# Autodesk Inventor assembly: 100008
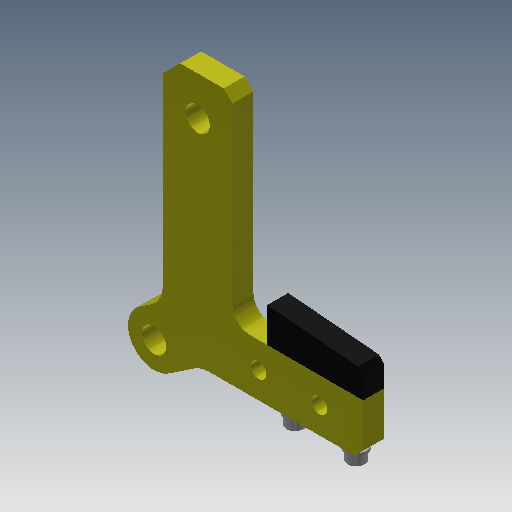
[picture p0: Inventor's stored thumbnail of the model, 512x512]
Saved by Autodesk Inventor 2020.1 (Build 241239000, 239)
## iProperties
Company: AUTODESK, INC.
Part Number: 100008
Document SubType Name: Assembly
Created: 2004-04-01
Designer: SCHNEIDER K.
Project: ADSK-000-000000
Description: CLAMP UNIT REAR FINGER
Control State: 0
Master: False
Checked Out: False
Shininess: 64.0
Length Units: 11269
Angle Units: 11279
Time Units: 11290
Mass Units: 11283
Length Display Precision: 3
Angle Display Precision: 2
Compacted: True
Density: 0.0
Volumn: 0.0
Area: 0.0
PropertySet Name: Model Information
Title: ASSEMBLY
Author: SCHNEIDER K.
Revision Number: -
## Documents named in this file (5)
- C:\Users\thom_tremblay\Desktop\Inventor ACP Data\Assemblies\210-103b.iam
- C:\Users\thom_tremblay\Desktop\Inventor ACP Data\Parts\210-104.ipt
- C:\Users\thom_tremblay\Desktop\Inventor ACP Data\Parts\210-105.ipt
- C:\Users\thom_tremblay\Desktop\Inventor ACP Data\Content Center\en-US\ISO 7089\6.ipt
- C:\Users\thom_tremblay\Desktop\Inventor ACP Data\Content Center\en-US\ISO 4762\M6-45.ipt
## Components (6 placed, 4 different names)
1. 210-104:1 — Mate:19, Mate:20, Mate:43, Insert:6, Insert:7
2. 210-105:1 — Mate:19, Mate:20, Mate:43
3. "ISO 7089" 6 - 140 HV:1 — Insert:5, Insert:6
4. "ISO 7089" 6 - 140 HV:2 — Insert:7, Insert:8
5. "ISO 4762 " M6 x 45:1 — Insert:5
6. "ISO 4762 " M6 x 45:2 — Insert:8
## Relationships (7: Insert 4, Mate 3)
- Mate:19: 210-104:1 ↔ 210-105:1
- Mate:20: 210-104:1 ↔ 210-105:1
- Mate:43: 210-104:1 ↔ 210-105:1
- Insert:5: "ISO 7089" 6 - 140 HV:1 ↔ "ISO 4762 " M6 x 45:1
- Insert:6: 210-104:1 ↔ "ISO 7089" 6 - 140 HV:1
- Insert:7: 210-104:1 ↔ "ISO 7089" 6 - 140 HV:2
- Insert:8: "ISO 7089" 6 - 140 HV:2 ↔ "ISO 4762 " M6 x 45:2
